# Autodesk Inventor assembly: LER_shooter
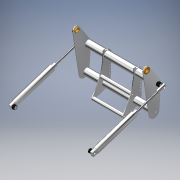
[picture p0: Inventor's stored thumbnail of the model, 180x180]
Saved by Autodesk Inventor 2019 (Build 230136000, 136)
## iProperties
Created: 2018-10-31
Part Number: LER_shooter
Document SubType Name: Assembly
Designer: woodk
Author: woodk
Revision Number: ANY
## Documents named in this file (12)
- F:\adrian-frc-team-1678-2016-1.snapshot.20\LER_shooter.iam
- F:\adrian-frc-team-1678-2016-1.snapshot.20\bushing_.5.ipt
- F:\adrian-frc-team-1678-2016-1.snapshot.20\1678-16-P-0905.ipt
- F:\adrian-frc-team-1678-2016-1.snapshot.20\pneumatic_.75x3.iam
- F:\adrian-frc-team-1678-2016-1.snapshot.20\1678-16-P-0907.ipt
- F:\adrian-frc-team-1678-2016-1.snapshot.20\1678-16-P-0908.ipt
- F:\adrian-frc-team-1678-2016-1.snapshot.20\1678-16-P-0913.ipt
- F:\adrian-frc-team-1678-2016-1.snapshot.20\1678-16-P-0914.ipt
- F:\adrian-frc-team-1678-2016-1.snapshot.20\1678-16-P-0915.ipt
- F:\adrian-frc-team-1678-2016-1.snapshot.20\1678-16-P-0916.ipt
- F:\adrian-frc-team-1678-2016-1.snapshot.20\1678-16-P-0912-rev1.ipt
- F:\adrian-frc-team-1678-2016-1.snapshot.20\LER shooter hood plate.ipt
## Components (26 placed, 26 different names)
1. 1678-16-P-0902_205 — Insert:1, Insert:3, Insert:7, Insert:10, Mate:5
2. bushing_.5_206 — Insert:1
3. bushing_.5_207 — Insert:11
4. 1678-16-P-0905_208 — Insert:14, Mate:2, Mate:7
5. pneumatic_.75x3_209 [sub-assembly] — Insert:14, Insert:16
6. 1678-16-P-0905_210 — Insert:2, Mate:1, Mate:6
7. 1678-16-P-0907_211 — Insert:16
8. 1678-16-P-0907_212 — Insert:4
9. 1678-16-P-0908_213 — Insert:15, Mate:2, Mate:7
10. 1678-16-P-0908_214 — Insert:3, Mate:1, Mate:6
11. 1678-16-P-0902_216 — Insert:11, Insert:12, Insert:13, Insert:15
12. 1678-16-P-0913_217 — Insert:5, Insert:6, Mate:8
13. 1678-16-P-0914_218 — Insert:17, Insert:18
14. 1678-16-P-0914_219 — Insert:20, Insert:21
15. pneumatic_.75x3_220 [sub-assembly] — Insert:2, Insert:4
16. 1678-16-P-0913_221 — Insert:8, Insert:9, Mate:4
17. 1678-16-P-0915_222 — Insert:6, Insert:12
18. 1678-16-P-0915_223 — Insert:8, Insert:10
19. 1678-16-P-0915_224 — Insert:5, Insert:7
20. 1678-16-P-0915_225 — Insert:9, Insert:13
21. 1678-16-P-0916_226 — Insert:17, Insert:19
22. 1678-16-P-0916_227 — Insert:21, Insert:23
23. 1678-16-P-0916_228 — Insert:18, Insert:24
24. 1678-16-P-0916_229 — Insert:20, Insert:22
25. 1678-16-P-0912-rev1_230 — Insert:19, Insert:22
26. 1678-16-P-0912-rev1_231 — Insert:23, Insert:24, Mate:4, Mate:5, Mate:8
## Relationships (31: Insert 24, Mate 7)
- Insert:1: 1678-16-P-0902_205 ↔ bushing_.5_206
- Insert:2 (-6.985 mm): 1678-16-P-0905_210 ↔ pneumatic_.75x3_220
- Insert:3: 1678-16-P-0902_205 ↔ 1678-16-P-0908_214
- Mate:1: 1678-16-P-0905_210 ↔ 1678-16-P-0908_214
- Insert:4: 1678-16-P-0907_212 ↔ pneumatic_.75x3_220
- Insert:5: 1678-16-P-0913_217 ↔ 1678-16-P-0915_224
- Insert:6: 1678-16-P-0913_217 ↔ 1678-16-P-0915_222
- Insert:7 (2.032 mm): 1678-16-P-0902_205 ↔ 1678-16-P-0915_224
- Insert:8: 1678-16-P-0913_221 ↔ 1678-16-P-0915_223
- Insert:9: 1678-16-P-0913_221 ↔ 1678-16-P-0915_225
- Insert:10 (2.032 mm): 1678-16-P-0902_205 ↔ 1678-16-P-0915_223
- Insert:11: bushing_.5_207 ↔ 1678-16-P-0902_216
- Insert:12 (2.032 mm): 1678-16-P-0902_216 ↔ 1678-16-P-0915_222
- Insert:13 (2.032 mm): 1678-16-P-0902_216 ↔ 1678-16-P-0915_225
- Insert:14 (-6.985 mm): 1678-16-P-0905_208 ↔ pneumatic_.75x3_209
- Insert:15: 1678-16-P-0908_213 ↔ 1678-16-P-0902_216
- Mate:2: 1678-16-P-0905_208 ↔ 1678-16-P-0908_213
- Insert:16: pneumatic_.75x3_209 ↔ 1678-16-P-0907_211
- Insert:17: 1678-16-P-0914_218 ↔ 1678-16-P-0916_226
- Insert:18: 1678-16-P-0914_218 ↔ 1678-16-P-0916_228
- Insert:19: 1678-16-P-0916_226 ↔ 1678-16-P-0912-rev1_230
- Insert:20: 1678-16-P-0914_219 ↔ 1678-16-P-0916_229
- Insert:21: 1678-16-P-0914_219 ↔ 1678-16-P-0916_227
- Insert:22: 1678-16-P-0916_229 ↔ 1678-16-P-0912-rev1_230
- Insert:23: 1678-16-P-0916_227 ↔ 1678-16-P-0912-rev1_231
- Insert:24: 1678-16-P-0916_228 ↔ 1678-16-P-0912-rev1_231
- Mate:4: 1678-16-P-0913_221 ↔ 1678-16-P-0912-rev1_231
- Mate:5 (72.136 mm): 1678-16-P-0902_205 ↔ 1678-16-P-0912-rev1_231
- Mate:6 (8.128 mm): 1678-16-P-0905_210 ↔ 1678-16-P-0908_214
- Mate:7 (8.128 mm): 1678-16-P-0905_208 ↔ 1678-16-P-0908_213
- Mate:8: 1678-16-P-0913_217 ↔ 1678-16-P-0912-rev1_231
